# Autodesk Inventor assembly: ABD_MX_64_Roll_Fixation_Set
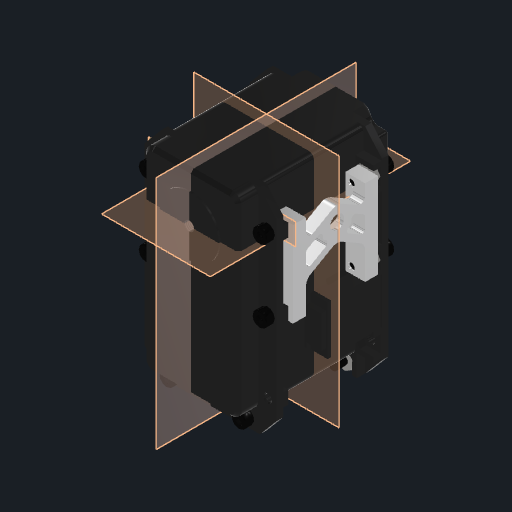
[picture p0: Inventor's stored thumbnail of the model, 512x512]
Saved by Autodesk Inventor 2024.3 (Build 283343000, 343)
## iProperties
Created: 2024-02-15
Part Number: ABD_MX_64_Roll_Fixation_Set
Document SubType Name: Assembly
Designer: ASUS
Author: ASUS
## Documents named in this file (5)
- C:\Users\ASUS\Desktop\Anti_Backlash_Structure_OP\v2_Frame\ABD_MX_64_Roll_Fixation_Set.iam
- C:\Users\ASUS\Desktop\ABD_2024_Eindhoven\MISUMI\Roll_Fixation_Frame_8mm_Set.iam
- C:\Users\ASUS\Desktop\Anti_Backlash_Structure_OP\v2_Frame\Roll_Fixation_L.ipt
- C:\Users\ASUS\Desktop\Anti_Backlash_Structure_OP\v2_Frame\Roll_Fixation_R.ipt
- C:\Users\ASUS\Desktop\Anti_Backlash_Structure_OP\ROBOTIS(Inventor 2024 ver.)\DXL\MX-106T.ipt
## Components (6 placed, 4 different names)
1. Roll_Fixation_Frame_8mm_Set:1 [sub-assembly] — 메이트:6, 메이트:7, 삽입:2, 메이트:15
2. Roll_Fixation_R:1 — 플러쉬:1, 메이트:8, 메이트:9, 메이트:11
3. Roll_Fixation_Frame_8mm_Set:2 [sub-assembly] — 메이트:8, 메이트:9, 삽입:1, 메이트:10
4. Roll_Fixation_L:1 — 메이트:6, 메이트:7, 플러쉬:1, 메이트:12, 메이트:13, 메이트:14
5. Roll_Fixation_Frame_8mm_Set:3 [sub-assembly] — 삽입:3, 메이트:16
6. MX-106T:1 — 삽입:1, 메이트:10, 메이트:11, 메이트:12, 메이트:13, 메이트:14, 삽입:2, 메이트:15, 삽입:3, 메이트:16
## Relationships (15: Mate 11, Insert 3, Flush 1)
- 메이트:6 [Mate]: Roll_Fixation_Frame_8mm_Set:1 ↔ Roll_Fixation_L:1
- 메이트:7 [Mate]: Roll_Fixation_Frame_8mm_Set:1 ↔ Roll_Fixation_L:1
- 플러쉬:1 [Flush]: Roll_Fixation_R:1 ↔ Roll_Fixation_L:1
- 메이트:8 [Mate]: Roll_Fixation_R:1 ↔ Roll_Fixation_Frame_8mm_Set:2
- 메이트:9 [Mate]: Roll_Fixation_R:1 ↔ Roll_Fixation_Frame_8mm_Set:2
- 삽입:1 [Insert]: Roll_Fixation_Frame_8mm_Set:2 ↔ MX-106T:1
- 메이트:10 [Mate]: Roll_Fixation_Frame_8mm_Set:2 ↔ MX-106T:1
- 메이트:11 [Mate] (0.05 mm): Roll_Fixation_R:1 ↔ MX-106T:1
- 메이트:12 [Mate] (0.05 mm): Roll_Fixation_L:1 ↔ MX-106T:1
- 메이트:13 [Mate]: Roll_Fixation_L:1 ↔ MX-106T:1
- 메이트:14 [Mate]: Roll_Fixation_L:1 ↔ MX-106T:1
- 삽입:2 [Insert]: Roll_Fixation_Frame_8mm_Set:1 ↔ MX-106T:1
- 메이트:15 [Mate]: Roll_Fixation_Frame_8mm_Set:1 ↔ MX-106T:1
- 삽입:3 [Insert]: Roll_Fixation_Frame_8mm_Set:3 ↔ MX-106T:1
- 메이트:16 [Mate]: Roll_Fixation_Frame_8mm_Set:3 ↔ MX-106T:1
